# Autodesk Inventor assembly: 08-04-00-000_clutchPaddleAssembly
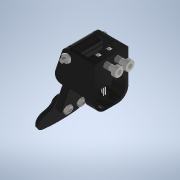
[picture p0: Inventor's stored thumbnail of the model, 180x180]
Saved by Autodesk Inventor 2020 (Build 240168000, 168)
## iProperties
Created: 2021-07-31
Part Number: 08-04-00-000_clutchPaddleAssembly
Document SubType Name: Assembly
Designer: Eric
Author: Eric
## Documents named in this file (12)
- C:\Users\Eric\Documents\repos\DIY_CAD_WheelButtonPlate\CAD\Inventor\08-04-00-000_clutchPaddleAssembly.iam
- C:\Users\Eric\Documents\repos\DIY_CAD_WheelButtonPlate\CAD\Inventor\08-04-01-002_clutchPaddleBase.ipt
- C:\Users\Eric\Documents\repos\DIY_CAD_WheelButtonPlate\CAD\Inventor\08-04-01-003_clutchPaddleLever.ipt
- C:\Users\Eric\Documents\Inventor\Content Center Files\R2020\de-DE\ISO 4032(1)\ISO 4032 - M4DIN EN.ipt
- C:\Users\Eric\Documents\Inventor\Content Center Files\R2020\de-DE\DIN 7991(2)\DIN 7991 - M3x10.ipt
- C:\Users\Eric\Documents\Inventor\Content Center Files\R2020\de-DE\ISO 4032(1)\ISO 4032 - M3DIN EN.ipt
- C:\Users\Eric\Documents\repos\DIY_CAD_WheelButtonPlate\CAD\Inventor\08-04-01-007_magnet15x3.ipt
- C:\Users\Eric\Documents\Inventor\Content Center Files\R2020\de-DE\DIN 6912\DIN 6912 - M4 x 16.ipt
- C:\Users\Eric\Documents\repos\DIY_CAD_WheelButtonPlate\CAD\Inventor\08-04-02-008_hallSensor.ipt
- C:\Users\Eric\Documents\Inventor\Content Center Files\R2020\de-DE\ISO 4762(1)\DIN EN ISO 4762 - M3 x 30.ipt
- C:\Users\Eric\Documents\repos\DIY_CAD_WheelButtonPlate\CAD\Inventor\08-04-01-006_clutchPaddle.ipt
- C:\Users\Eric\Documents\repos\DIY_CAD_WheelButtonPlate\CAD\Inventor\08-04-02-004_magnet12x3.ipt
## Components (17 placed, 11 different names)
1. 08-04-01-002_clutchPaddleBase:1 — Passend:1, Passend:2, Passend:5, Passend:26, Passend:27, Passend:33, Passend:35, Einfügen:2, Einfügen:3, Passend:36, Passend:37, Fluchtend:3, Fluchtend:4, Passend:38, Passend:39, Passend:40, Einfügen:4, Passend:41
2. 08-04-01-003_clutchPaddleLever:1 — Passend:1, Passend:2, Passend:24, Passend:25, Passend:28, Passend:29, Fluchtend:1, Fluchtend:2, Passend:31, Passend:32, Passend:41, Passend:42, Passend:45, Passend:46
3. DIN EN 24032 M3:5 — Passend:5
4. DIN 7991 M3x10:4 — Passend:22, Fluchtend:1, Passend:32, Passend:43
5. DIN 7991 M3x10:5 — Passend:23, Fluchtend:2, Passend:31, Passend:44
6. DIN EN 24032 M3:3 — Passend:23, Passend:24
7. DIN EN 24032 M3:4 — Passend:22, Passend:25
8. 08-04-01-007_magnet15x3:1 — Passend:26, Passend:27
9. 08-04-01-007_magnet15x3:2 — Passend:28, Passend:29
10. DIN 6912 M4 x 16:1 — Passend:33, Fluchtend:3
11. DIN 6912 M4 x 16:2 — Passend:35, Fluchtend:4
12. DIN EN 24032 M4:2 — Einfügen:2, Passend:36
13. DIN EN 24032 M4:3 — Einfügen:3, Passend:37
14. 08-04-02-008_hallSensor_49E:1 — Passend:38, Passend:39, Passend:40
15. DIN EN ISO 4762 M3 x 30:1 — Einfügen:4
16. 08-04-01-006_clutchPaddle:1 — Passend:42, Passend:43, Passend:44
17. 08-04-02-004_magnet12x3:1 — Passend:45, Passend:46
## Relationships (33: Mate 26, Flush 4, Insert 3)
- Passend:1 [Mate]: 08-04-01-002_clutchPaddleBase:1 ↔ 08-04-01-003_clutchPaddleLever:1
- Passend:2 [Mate] (0.4 mm): 08-04-01-002_clutchPaddleBase:1 ↔ 08-04-01-003_clutchPaddleLever:1
- Passend:5 [Mate]: 08-04-01-002_clutchPaddleBase:1 ↔ DIN EN 24032 M3:5
- Passend:22 [Mate]: DIN 7991 M3x10:4 ↔ DIN EN 24032 M3:4
- Passend:23 [Mate]: DIN 7991 M3x10:5 ↔ DIN EN 24032 M3:3
- Passend:24 [Mate]: 08-04-01-003_clutchPaddleLever:1 ↔ DIN EN 24032 M3:3
- Passend:25 [Mate]: 08-04-01-003_clutchPaddleLever:1 ↔ DIN EN 24032 M3:4
- Passend:26 [Mate]: 08-04-01-002_clutchPaddleBase:1 ↔ 08-04-01-007_magnet15x3:1
- Passend:27 [Mate]: 08-04-01-002_clutchPaddleBase:1 ↔ 08-04-01-007_magnet15x3:1
- Passend:28 [Mate]: 08-04-01-003_clutchPaddleLever:1 ↔ 08-04-01-007_magnet15x3:2
- Passend:29 [Mate]: 08-04-01-003_clutchPaddleLever:1 ↔ 08-04-01-007_magnet15x3:2
- Fluchtend:1 [Flush] (-3.1 mm): 08-04-01-003_clutchPaddleLever:1 ↔ DIN 7991 M3x10:4
- Fluchtend:2 [Flush] (-3.1 mm): 08-04-01-003_clutchPaddleLever:1 ↔ DIN 7991 M3x10:5
- Passend:31 [Mate]: 08-04-01-003_clutchPaddleLever:1 ↔ DIN 7991 M3x10:5
- Passend:32 [Mate]: 08-04-01-003_clutchPaddleLever:1 ↔ DIN 7991 M3x10:4
- Passend:33 [Mate]: 08-04-01-002_clutchPaddleBase:1 ↔ DIN 6912 M4 x 16:1
- Passend:35 [Mate]: 08-04-01-002_clutchPaddleBase:1 ↔ DIN 6912 M4 x 16:2
- Einfügen:2 [Insert]: 08-04-01-002_clutchPaddleBase:1 ↔ DIN EN 24032 M4:2
- Einfügen:3 [Insert]: 08-04-01-002_clutchPaddleBase:1 ↔ DIN EN 24032 M4:3
- Passend:36 [Mate]: 08-04-01-002_clutchPaddleBase:1 ↔ DIN EN 24032 M4:2
- Passend:37 [Mate]: 08-04-01-002_clutchPaddleBase:1 ↔ DIN EN 24032 M4:3
- Fluchtend:3 [Flush] (15 mm): 08-04-01-002_clutchPaddleBase:1 ↔ DIN 6912 M4 x 16:1
- Fluchtend:4 [Flush] (15 mm): 08-04-01-002_clutchPaddleBase:1 ↔ DIN 6912 M4 x 16:2
- Passend:38 [Mate]: 08-04-01-002_clutchPaddleBase:1 ↔ 08-04-02-008_hallSensor_49E:1
- Passend:39 [Mate]: 08-04-01-002_clutchPaddleBase:1 ↔ 08-04-02-008_hallSensor_49E:1
- Passend:40 [Mate]: 08-04-01-002_clutchPaddleBase:1 ↔ 08-04-02-008_hallSensor_49E:1
- Einfügen:4 [Insert]: 08-04-01-002_clutchPaddleBase:1 ↔ DIN EN ISO 4762 M3 x 30:1
- Passend:41 [Mate]: 08-04-01-002_clutchPaddleBase:1 ↔ 08-04-01-003_clutchPaddleLever:1
- Passend:42 [Mate]: 08-04-01-003_clutchPaddleLever:1 ↔ 08-04-01-006_clutchPaddle:1
- Passend:43 [Mate]: DIN 7991 M3x10:4 ↔ 08-04-01-006_clutchPaddle:1
- Passend:44 [Mate]: DIN 7991 M3x10:5 ↔ 08-04-01-006_clutchPaddle:1
- Passend:45 [Mate]: 08-04-01-003_clutchPaddleLever:1 ↔ 08-04-02-004_magnet12x3:1
- Passend:46 [Mate]: 08-04-01-003_clutchPaddleLever:1 ↔ 08-04-02-004_magnet12x3:1
